# Autodesk Inventor assembly: MONTAGEM DO BOTÃO
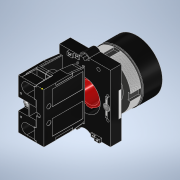
[picture p0: Inventor's stored thumbnail of the model, 180x180]
Saved by Autodesk Inventor 2022 (Build 260153000, 153)
## iProperties
Created: 2023-07-20
Part Number: MONTAGEM DO BOTÃO
Document SubType Name: Assembly
Designer: Usuário
Author: Usuário
## Documents named in this file (8)
- G:\Meu Drive\PROJETOS INTERNOS22\PLATAFORMA ELEVATORIA\22.08_PLATAFORMA_PLATAFORMA COMPLETA-IGARASSU-PE.R00\PROJETOS\MODELAGEM\PEÇAS HIDRAULICA-ELETRONICA\BOTÃO LK2-EA42 (VERMELHO) 1NF CÓD 14010\MONTAGEM DO BOTÃO.iam
- G:\Meu Drive\PROJETOS INTERNOS22\PLATAFORMA ELEVATORIA\22.08_PLATAFORMA_PLATAFORMA COMPLETA-IGARASSU-PE.R00\PROJETOS\MODELAGEM\PEÇAS HIDRAULICA-ELETRONICA\BOTÃO LK2-EA42 (VERMELHO) 1NF CÓD 14010\BASE DO BOTÃO LK-2EA42 .ipt
- G:\Meu Drive\PROJETOS INTERNOS22\PLATAFORMA ELEVATORIA\22.08_PLATAFORMA_PLATAFORMA COMPLETA-IGARASSU-PE.R00\PROJETOS\MODELAGEM\PEÇAS HIDRAULICA-ELETRONICA\BOTÃO LK2-EA42 (VERMELHO) 1NF CÓD 14010\BOTÃO.ipt
- G:\Meu Drive\PROJETOS INTERNOS22\PLATAFORMA ELEVATORIA\22.08_PLATAFORMA_PLATAFORMA COMPLETA-IGARASSU-PE.R00\PROJETOS\MODELAGEM\PEÇAS HIDRAULICA-ELETRONICA\BOTÃO LK2-EA42 (VERMELHO) 1NF CÓD 14010\PORCA2.ipt
- G:\Meu Drive\PROJETOS INTERNOS22\PLATAFORMA ELEVATORIA\22.08_PLATAFORMA_PLATAFORMA COMPLETA-IGARASSU-PE.R00\PROJETOS\MODELAGEM\PEÇAS HIDRAULICA-ELETRONICA\BOTÃO LK2-EA42 (VERMELHO) 1NF CÓD 14010\ARRUELA2.ipt
- G:\Meu Drive\PROJETOS INTERNOS22\PLATAFORMA ELEVATORIA\22.08_PLATAFORMA_PLATAFORMA COMPLETA-IGARASSU-PE.R00\PROJETOS\MODELAGEM\PEÇAS HIDRAULICA-ELETRONICA\BOTÃO LK2-EA42 (VERMELHO) 1NF CÓD 14010\fixação do pino.ipt
- G:\Meu Drive\PROJETOS INTERNOS22\PLATAFORMA ELEVATORIA\22.08_PLATAFORMA_PLATAFORMA COMPLETA-IGARASSU-PE.R00\PROJETOS\MODELAGEM\PEÇAS HIDRAULICA-ELETRONICA\BOTÃO LK2-EA42 (VERMELHO) 1NF CÓD 14010\bloco de contato vermelho.ipt
- G:\Meu Drive\PROJETOS INTERNOS22\PLATAFORMA ELEVATORIA\22.08_PLATAFORMA_PLATAFORMA COMPLETA-IGARASSU-PE.R00\PROJETOS\MODELAGEM\PEÇAS HIDRAULICA-ELETRONICA\BOTÃO LK2-EA42 (VERMELHO) 1NF CÓD 14010\PINO DO BLOCO DE CONTATO.ipt
## Components (8 placed, 7 different names)
1. BASE DO BOTÃO LK-2EA42 :1 — Mate:1, Flush:1, Mate:2, Mate:3, Mate:4, Mate:6, Mate:7, Mate:8, Mate:9, Angle:1, Mate:11
2. BOTÃO:1 — Mate:1, Flush:1
3. PORCA2:1 — Mate:2, Mate:5
4. ARRUELA2:1 — Mate:3, Mate:4, Mate:5
5. fixação do pino:1 — Mate:6, Mate:7
6. fixação do pino:2 — Mate:8, Mate:9, Mate:10
7. bloco de contato vermelho:1 — Mate:10, Angle:1, Mate:11, Mate:12, Mate:13
8. PINO DO BLOCO DE CONTATO:1 — Mate:12, Mate:13
## Relationships (15: Mate 13, Flush 1, Angle 1)
- Mate:1: BASE DO BOTÃO LK-2EA42 :1 ↔ BOTÃO:1
- Flush:1: BASE DO BOTÃO LK-2EA42 :1 ↔ BOTÃO:1
- Mate:2: BASE DO BOTÃO LK-2EA42 :1 ↔ PORCA2:1
- Mate:3: BASE DO BOTÃO LK-2EA42 :1 ↔ ARRUELA2:1
- Mate:4: BASE DO BOTÃO LK-2EA42 :1 ↔ ARRUELA2:1
- Mate:5: PORCA2:1 ↔ ARRUELA2:1
- Mate:6: BASE DO BOTÃO LK-2EA42 :1 ↔ fixação do pino:1
- Mate:7: BASE DO BOTÃO LK-2EA42 :1 ↔ fixação do pino:1
- Mate:8: BASE DO BOTÃO LK-2EA42 :1 ↔ fixação do pino:2
- Mate:9: BASE DO BOTÃO LK-2EA42 :1 ↔ fixação do pino:2
- Mate:10: fixação do pino:2 ↔ bloco de contato vermelho:1
- Angle:1 (0 deg): BASE DO BOTÃO LK-2EA42 :1 ↔ bloco de contato vermelho:1
- Mate:11: BASE DO BOTÃO LK-2EA42 :1 ↔ bloco de contato vermelho:1
- Mate:12: bloco de contato vermelho:1 ↔ PINO DO BLOCO DE CONTATO:1
- Mate:13: bloco de contato vermelho:1 ↔ PINO DO BLOCO DE CONTATO:1
